# Autodesk Inventor assembly: Assembly1
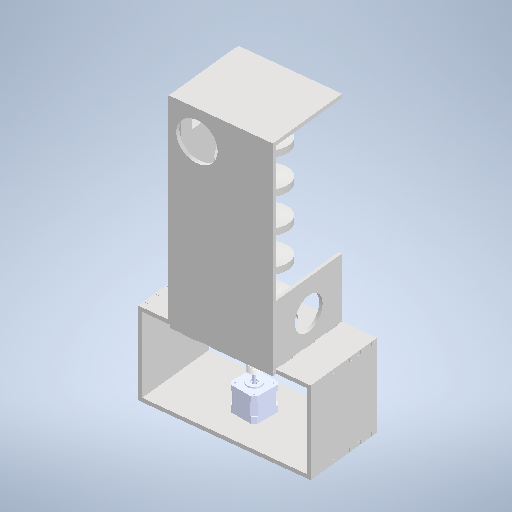
[picture p0: Inventor's stored thumbnail of the model, 512x512]
Saved by Autodesk Inventor 2025.3 (Build 293356000, 356)
## iProperties
Created: 2026-04-14
Part Number: Assembly1
Document SubType Name: Assembly
Designer: ziada
Author: ziada
## Documents named in this file (12)
- C:\Sophomore\Semester 4\Basics of Mechatronics\BOM Project\Assembly1.iam
- C:\Sophomore\Semester 4\Basics of Mechatronics\BOM Project\NEMA17 Model STEP\NEMA17 Model STEP\NEMA17 Model STEP.iam
- C:\Sophomore\Semester 4\Basics of Mechatronics\BOM Project\Flexible Shaft Coupler 5x8mm\Flexible Shaft Coupler 5x8mm\Flexible Shaft Coupler 5x8mm.ipt
- C:\Sophomore\Semester 4\Basics of Mechatronics\BOM Project\Archimedes Screw V2.ipt
- C:\Sophomore\Semester 4\Basics of Mechatronics\BOM Project\Insert.ipt
- C:\Sophomore\Semester 4\Basics of Mechatronics\BOM Project\Base.ipt
- C:\Sophomore\Semester 4\Basics of Mechatronics\BOM Project\Wall.ipt
- C:\Sophomore\Semester 4\Basics of Mechatronics\BOM Project\Top.ipt
- C:\Sophomore\Semester 4\Basics of Mechatronics\BOM Project\Wall2.ipt
- C:\Sophomore\Semester 4\Basics of Mechatronics\BOM Project\Exit.ipt
- C:\Sophomore\Semester 4\Basics of Mechatronics\BOM Project\Base2.ipt
- C:\Sophomore\Semester 4\Basics of Mechatronics\BOM Project\Base Connection.ipt
## Components (12 placed, 11 different names)
1. NEMA17 Model STEP:1 [sub-assembly] — Insert:1
2. Flexible Shaft Coupler 5x8mm:1 — Insert:1, Insert:2
3. Archimedes Screw V2:1 — Insert:2, Insert:3
4. Base:1 — Insert:3, Mate:3, Mate:4, Mate:5, Mate:6, Mate:8, Mate:9, Mate:12, Mate:13, Mate:14, Mate:15, Mate:18, Mate:19
5. Top:1 — Mate:20, Mate:21
6. Wall:1 — Mate:3, Mate:4, Mate:7
7. Wall2:1 — Mate:5, Mate:6, Mate:7, Mate:21
8. Exit:1 — Mate:8, Mate:9, Mate:20
9. Base2:1 — Mate:16, Mate:17
10. Base Connection:1 — Mate:12, Mate:13
11. Base Connection:2 — Mate:14, Mate:15, Mate:16, Mate:17
12. Insert:1 — Mate:18, Mate:19
## Relationships (20: Mate 17, Insert 3)
- Insert:1 (-5 mm): NEMA17 Model STEP:1 ↔ Flexible Shaft Coupler 5x8mm:1
- Insert:2 (-5 mm): Flexible Shaft Coupler 5x8mm:1 ↔ Archimedes Screw V2:1
- Insert:3 (-15 mm): Archimedes Screw V2:1 ↔ Base:1
- Mate:3: Base:1 ↔ Wall:1
- Mate:4: Base:1 ↔ Wall:1
- Mate:5: Base:1 ↔ Wall2:1
- Mate:6: Base:1 ↔ Wall2:1
- Mate:7: Wall:1 ↔ Wall2:1
- Mate:8: Base:1 ↔ Exit:1
- Mate:9: Base:1 ↔ Exit:1
- Mate:12: Base:1 ↔ Base Connection:1
- Mate:13: Base:1 ↔ Base Connection:1
- Mate:14: Base:1 ↔ Base Connection:2
- Mate:15: Base:1 ↔ Base Connection:2
- Mate:16: Base2:1 ↔ Base Connection:2
- Mate:17: Base2:1 ↔ Base Connection:2
- Mate:18: Base:1 ↔ Insert:1
- Mate:19: Base:1 ↔ Insert:1
- Mate:20: Top:1 ↔ Exit:1
- Mate:21: Top:1 ↔ Wall2:1
